# Autodesk Inventor assembly: Big_housing
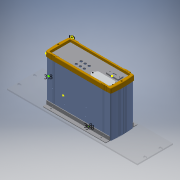
[picture p0: Inventor's stored thumbnail of the model, 180x180]
Saved by Autodesk Inventor 2018 (Build 220112000, 112)
## iProperties
Created: 2012-02-06
Part Number: Big_housing
Document SubType Name: Assembly
Designer: Huethe
Übersetzungsnorm: STEP AP214IS
Dateiname: 41800160.stp
Vorprozessor: OneSpace Modeling 15.50A  21-Sep-2007 (C) CoCreate Software GmbH
Postprozessor: Build: 223b, Release: 2010 RTM - Date: Sat 02/14/2009
Gesendete Einheiten: Millimeter
Unbestimmtheit: 1e-06
Author: Huethe
## Documents named in this file (12)
- C:\Users\David\Documents\optoelectronics\CAD\Bigdriver_box\Big_housing.iam
- C:\Users\David\Documents\optoelectronics\CAD\Bigdriver_box\Apra_X-dream_418\041800100_Blendrahmen_X_Dream_418.ipt
- C:\Users\David\Documents\optoelectronics\CAD\Bigdriver_box\Apra_X-dream_418\041800222_Profil_X_Dream_t220.1.ipt
- C:\Users\David\Documents\optoelectronics\CAD\Bigdriver_box\Apra_X-dream_418\Frontplatte_Apra_Xdream_418.ipt
- C:\Users\David\Documents\optoelectronics\CAD\Bigdriver_box\PCB.ipt
- C:\Users\David\Documents\optoelectronics\CAD\Bigdriver_box\Schurter_CDG4_4101_151.ipt
- C:\Users\David\Documents\optoelectronics\CAD\Bigdriver_box\source.ipt
- C:\Users\David\Documents\optoelectronics\CAD\usb-better-1.snapshot.4\usb head.ipt
- C:\Users\David\Documents\optoelectronics\CAD\usb-better-1.snapshot.4\USB_housing.ipt
- C:\Users\David\Documents\optoelectronics\CAD\Bigdriver_box\Apra_X-dream_418\Large_frontplatte.ipt
- C:\Users\David\Documents\optoelectronics\CAD\Bigdriver_box\Apra_X-dream_418\L.ipt
- C:\Users\David\Documents\optoelectronics\CAD\Bigdriver_box\Apra_X-dream_418\L_bottom.ipt
## Components (11 placed, 11 different names)
1. 041800100_Blendrahmen_X_Dream_418:1 — Mate:13, Mate:14, Angle:5
2. 041800222_Profil_X_Dream_t220.1:1 — Flush:4, Mate:28, Mate:29, Mate:30, Angle:6, Mate:32, Mate:33, Mate:34, Mate:36, Mate:37, Mate:38, Mate:39, Mate:42, Mate:44, Angle:8, Mate:45, Mate:46
3. Frontplatte_Apra_Xdream_418:3 — Mate:13, Mate:14, Angle:5, Mate:20, Mate:24, Mate:25, Mate:26, Mate:42, Mate:43, Angle:7, Mate:44, Angle:8
4. PCB:1 — Mate:45, Mate:46
5. Schurter_CDG4_4101_151:1 — Mate:20, Mate:43, Angle:7
6. source:1 — Flush:4, Mate:38, Mate:39
7. usb head:1 — Mate:21, Mate:22, Mate:23
8. USB_housing:1 — Mate:21, Mate:22, Mate:23, Mate:24, Mate:25, Mate:26
9. Large_frontplatte:1 — Mate:28, Mate:29, Mate:30, Angle:6, Mate:31, Mate:35
10. L:1 — Mate:31, Mate:32, Mate:33, Mate:34
11. L_bottom:1 — Mate:35, Mate:36, Mate:37
## Relationships (31: Mate 26, Angle 4, Flush 1)
- Mate:13: 041800100_Blendrahmen_X_Dream_418:1 ↔ Frontplatte_Apra_Xdream_418:3
- Mate:14: 041800100_Blendrahmen_X_Dream_418:1 ↔ Frontplatte_Apra_Xdream_418:3
- Angle:5 (0 deg): 041800100_Blendrahmen_X_Dream_418:1 ↔ Frontplatte_Apra_Xdream_418:3
- Flush:4 (2 mm): 041800222_Profil_X_Dream_t220.1:1 ↔ source:1
- Mate:20: Frontplatte_Apra_Xdream_418:3 ↔ Schurter_CDG4_4101_151:1
- Mate:21: usb head:1 ↔ USB_housing:1
- Mate:22: usb head:1 ↔ USB_housing:1
- Mate:23 (0.475 mm): usb head:1 ↔ USB_housing:1
- Mate:24: Frontplatte_Apra_Xdream_418:3 ↔ USB_housing:1
- Mate:25: Frontplatte_Apra_Xdream_418:3 ↔ USB_housing:1
- Mate:26: Frontplatte_Apra_Xdream_418:3 ↔ USB_housing:1
- Mate:28: 041800222_Profil_X_Dream_t220.1:1 ↔ Large_frontplatte:1
- Mate:29: 041800222_Profil_X_Dream_t220.1:1 ↔ Large_frontplatte:1
- Mate:30: 041800222_Profil_X_Dream_t220.1:1 ↔ Large_frontplatte:1
- Angle:6 (0 deg): 041800222_Profil_X_Dream_t220.1:1 ↔ Large_frontplatte:1
- Mate:31: Large_frontplatte:1 ↔ L:1
- Mate:32: 041800222_Profil_X_Dream_t220.1:1 ↔ L:1
- Mate:33: 041800222_Profil_X_Dream_t220.1:1 ↔ L:1
- Mate:34: 041800222_Profil_X_Dream_t220.1:1 ↔ L:1
- Mate:35: Large_frontplatte:1 ↔ L_bottom:1
- Mate:36: 041800222_Profil_X_Dream_t220.1:1 ↔ L_bottom:1
- Mate:37: 041800222_Profil_X_Dream_t220.1:1 ↔ L_bottom:1
- Mate:38: 041800222_Profil_X_Dream_t220.1:1 ↔ source:1
- Mate:39 (8 mm): 041800222_Profil_X_Dream_t220.1:1 ↔ source:1
- Mate:42: 041800222_Profil_X_Dream_t220.1:1 ↔ Frontplatte_Apra_Xdream_418:3
- Mate:43: Frontplatte_Apra_Xdream_418:3 ↔ Schurter_CDG4_4101_151:1
- Angle:7 (0 deg): Frontplatte_Apra_Xdream_418:3 ↔ Schurter_CDG4_4101_151:1
- Mate:44: 041800222_Profil_X_Dream_t220.1:1 ↔ Frontplatte_Apra_Xdream_418:3
- Angle:8 (0 deg): 041800222_Profil_X_Dream_t220.1:1 ↔ Frontplatte_Apra_Xdream_418:3
- Mate:45: 041800222_Profil_X_Dream_t220.1:1 ↔ PCB:1
- Mate:46 (10 mm): 041800222_Profil_X_Dream_t220.1:1 ↔ PCB:1
